# Autodesk Inventor assembly: Pannels Assembly
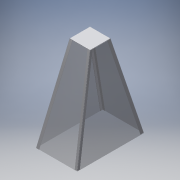
[picture p0: Inventor's stored thumbnail of the model, 180x180]
Saved by Autodesk Inventor 2016 (Build 200138000, 138)
## iProperties
Created: 2018-05-16
Part Number: Pannels Assembly
Document SubType Name: Assembly
Designer: Kade
Mass: 6944.74 g
Surface Area: 31644.1 cm^2
Volume: 4927.67 cm^3
Density: 1.40934 g/cm^3
Author: Kade
## Documents named in this file (6)
- F:\Robotics\Off Season\Blannon\Pannels Assembly.iam
- F:\Robotics\Off Season\Blannon\Polycarb Front Pannel.ipt
- F:\Robotics\Off Season\Blannon\Turntable Bottom.ipt
- F:\Robotics\Off Season\Blannon\Polycarb Back Pannel.ipt
- F:\Robotics\Off Season\Blannon\AngleL.ipt
- F:\Robotics\Off Season\Blannon\Polycarb Side1 Pannel.ipt
## Components (9 placed, 5 different names)
1. Turntable Bottom:1 — Flush:1, Mate:1, Mate:2, Mate:6, Mate:17, Mate:19
2. Polycarb Front Pannel:1 — Mate:6, Mate:14, Mate:18, Mate:21
3. Polycarb Back Pannel:1 — Mate:16, Mate:20, Mate:22, Mate:23
4. AngleL:1 — Mate:14
5. AngleL:2
6. AngleL:3 — Mate:16, Mate:22
7. AngleL:4
8. Polycarb Side1 Pannel:1 — Mate:17, Mate:18, Mate:23
9. Polycarb Side1 Pannel:2 — Mate:19, Mate:20, Mate:21
## Relationships (13: Mate 12, Flush 1)
- Flush:1: Turntable Bottom:1
- Mate:1 (-101.6 mm): Turntable Bottom:1
- Mate:2 (-101.6 mm): Turntable Bottom:1
- Mate:6: Turntable Bottom:1 ↔ Polycarb Front Pannel:1
- Mate:14: Polycarb Front Pannel:1 ↔ AngleL:1
- Mate:16: Polycarb Back Pannel:1 ↔ AngleL:3
- Mate:17: Turntable Bottom:1 ↔ Polycarb Side1 Pannel:1
- Mate:18: Polycarb Front Pannel:1 ↔ Polycarb Side1 Pannel:1
- Mate:19: Turntable Bottom:1 ↔ Polycarb Side1 Pannel:2
- Mate:20: Polycarb Back Pannel:1 ↔ Polycarb Side1 Pannel:2
- Mate:21: Polycarb Front Pannel:1 ↔ Polycarb Side1 Pannel:2
- Mate:22: Polycarb Back Pannel:1 ↔ AngleL:3
- Mate:23: Polycarb Back Pannel:1 ↔ Polycarb Side1 Pannel:1
